# Autodesk Inventor assembly: Assembly ss3
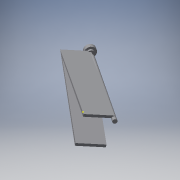
[picture p0: Inventor's stored thumbnail of the model, 180x180]
Saved by Autodesk Inventor 2019 (Build 230136000, 136)
## iProperties
Created: 2020-04-17
Part Number: Assembly ss3
Document SubType Name: Assembly
Designer: User
Author: User
## Documents named in this file (4)
- C:\Users\User\Desktop\assembly\Assembly ss2.iam
- C:\Users\User\Desktop\roller.ipt
- C:\Users\User\Desktop\motor.ipt
- C:\Users\User\Desktop\separator.ipt
## Components (3 placed, 3 different names)
1. roller:1 — Rotational:1, Rigid:1
2. motor:1 — Rotational:1
3. separator:1 — Rigid:1
## Relationships (2: RevoluteJoint 1, WeldJoint 1)
- Rotational:1 [RevoluteJoint]: roller:1 ↔ motor:1
- Rigid:1 [WeldJoint]: roller:1 ↔ separator:1
